# Autodesk Inventor assembly: aerogelInHolder
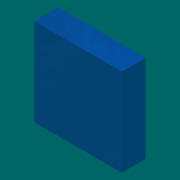
[picture p0: Inventor's stored thumbnail of the model, 180x180]
Saved by Autodesk Inventor 2016 (Build 200138000, 138)
## iProperties
Created: 2015-10-27
Part Number: aerogelInHolder
Document SubType Name: Assembly
Designer: Sawaiz
Author: Sawaiz
## Documents named in this file (4)
- C:\Users\Sawaiz\OneDrive\projects\modularRICH\aerogel\aerogelInHolder.iam
- C:\Users\Sawaiz\OneDrive\projects\modularRICH\aerogel\aerogelBlock.ipt
- C:\Users\Sawaiz\OneDrive\projects\modularRICH\aerogel\aerogelHolder.ipt
- C:\Users\Sawaiz\OneDrive\projects\modularRICH\modularRICH.xlsx
## Components (3 placed, 2 different names)
1. aerogelBlock:1 — Mate:1, Mate:2, Mate:3, Mate:4
2. aerogelHolder:1 — Flush:1, Flush:2, Mate:1, Mate:3
3. aerogelHolder:2 — Flush:1, Flush:2, Mate:2, Mate:4
## Relationships (6: Mate 4, Flush 2)
- Flush:1: aerogelHolder:1 ↔ aerogelHolder:2
- Flush:2: aerogelHolder:1 ↔ aerogelHolder:2
- Mate:1 (1.5875 mm): aerogelBlock:1 ↔ aerogelHolder:1
- Mate:2: aerogelBlock:1 ↔ aerogelHolder:2
- Mate:3: aerogelBlock:1 ↔ aerogelHolder:1
- Mate:4 (1.5875 mm): aerogelBlock:1 ↔ aerogelHolder:2
## Named parameters: frameAcrylicThickness = 9.525 mm, internalAcrylicThickness = 6.35 mm, aerogelThickness = 30 mm, aerogelWidth = 110 mm, aerogelHeight = 110 mm, height = 127 mm, width = 127 mm, depth = 273.05 mm, mirrorAngle = 5 deg, detectorWidth = 52 mm, detectorHeight = 52 mm, mirrorThickness = 3.175 mm, fresnelThickness = 0.1 mm, grooveDensity = 100, focalLength = 76.2 mm, ior = 1.49, centerThickness = 1.524 mm, fresnelAngle = 90 deg, fresnelEffectiveDiameter = 152.4 mm, oRingWidth = 1.5875 mm, sensorHolderDepth = 19.05 mm, aerogelClearence = 3.175 mm, backplaneHoleOffsett = 6.35 mm, backplanePCBWidth = 76.2 mm, backplanePCBHeight = 76.2 mm, backplanePostionOffsett = 12.7 mm, moduleSlotClearence = 0.79375 mm, testMountLength = 500 mm, testMountWidth = 300 mm, testMountHeight = 300 mm
